# Autodesk Inventor assembly: 15102898-16-A-0300
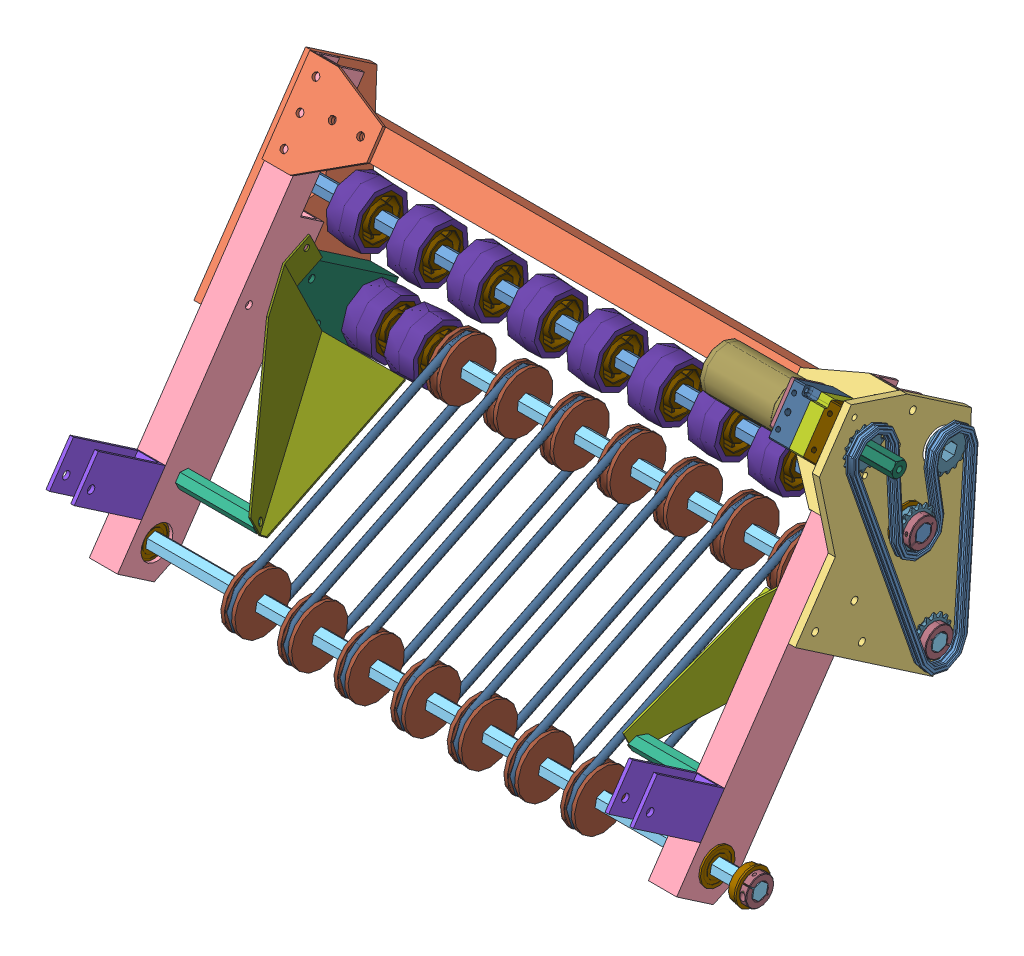
[picture p0: shaded view drawn from the shape stored in the file]
Saved by Autodesk Inventor 2017 (Build 210142000, 142)
## iProperties
Created: 2016-10-02
Part Number: 15102898-16-A-0300
Document SubType Name: Assembly
Designer: gus
Mass: 5609.92 g
Surface Area: 11678.6 cm^2
Volume: 2397.48 cm^3
Density: 2.33992 g/cm^3
Author: gus
## Documents named in this file (23)
- \\Mac\Home\Desktop\bunnybots 2016\15102898-16-Bunnybot-CAD\Bunnybot-To_be_renamed\15102898-16-A-0000\15102898-16-A-0300\15102898-16-A-0300.iam
- \\Mac\Home\Desktop\bunnybots 2016\15102898-16-Bunnybot-CAD\Bunnybot-To_be_renamed\15102898-16-A-0000\15102898-16-A-0300\15102898-16-P-0301.ipt
- \\Mac\Home\Desktop\bunnybots 2016\15102898-16-Bunnybot-CAD\Bunnybot-To_be_renamed\15102898-16-A-0000\15102898-16-A-0300\15102898-16-P-0302.ipt
- \\Mac\Home\Desktop\bunnybots 2016\15102898-16-Bunnybot-CAD\Bunnybot-To_be_renamed\15102898-16-A-0000\15102898-16-A-0300\Imported Components\217-3875-STEP-20140818.ipt
- \\Mac\Home\Desktop\bunnybots 2016\15102898-16-Bunnybot-CAD\Bunnybot-To_be_renamed\15102898-16-A-0000\15102898-16-A-0300\15102898-16-P-0303.ipt
- \\Mac\Home\Desktop\bunnybots 2016\15102898-16-Bunnybot-CAD\Bunnybot-To_be_renamed\15102898-16-A-0000\15102898-16-A-0300\Imported Components\217-2737.20121205.ipt
- \\Mac\Home\Desktop\bunnybots 2016\15102898-16-Bunnybot-CAD\Bunnybot-To_be_renamed\15102898-16-A-0000\15102898-16-A-0300\15102898-16-P-0304.ipt
- \\Mac\Home\Desktop\bunnybots 2016\15102898-16-Bunnybot-CAD\Bunnybot-To_be_renamed\15102898-16-A-0000\15102898-16-A-0300\15102898-16-P-0305.ipt
- \\Mac\Home\Desktop\bunnybots 2016\15102898-16-Bunnybot-CAD\Bunnybot-To_be_renamed\15102898-16-A-0000\15102898-16-A-0300\Imported Components\217-2642-STEP-20140807.ipt
- \\Mac\Home\Desktop\bunnybots 2016\15102898-16-Bunnybot-CAD\Bunnybot-To_be_renamed\15102898-16-A-0000\15102898-16-A-0300\Imported Components\BAG motor\VersaPlanetary-1-Stage-with-BAG-Motor.iam
- \\Mac\Home\Desktop\bunnybots 2016\15102898-16-Bunnybot-CAD\Bunnybot-To_be_renamed\15102898-16-A-0000\15102898-16-A-0300\Imported Components\6284K520_ROUND-BELT PULLEY.ipt
- \\Mac\Home\Desktop\bunnybots 2016\15102898-16-Bunnybot-CAD\Bunnybot-To_be_renamed\15102898-16-A-0000\15102898-16-A-0300\15102898-16-P-0308.ipt
- \\Mac\Home\Desktop\bunnybots 2016\15102898-16-Bunnybot-CAD\Bunnybot-To_be_renamed\15102898-16-A-0000\15102898-16-A-0300\Imported Components\am-3155+2in+Wheel+Intergrated+500+HEX.ipt
- \\Mac\Home\Desktop\bunnybots 2016\15102898-16-Bunnybot-CAD\Bunnybot-To_be_renamed\15102898-16-A-0000\15102898-16-A-0300\15102898-16-P-0307.ipt
- \\Mac\Home\Desktop\bunnybots 2016\15102898-16-Bunnybot-CAD\Bunnybot-To_be_renamed\15102898-16-A-0000\15102898-16-A-0300\15102898-16-P-0309.ipt
- \\Mac\Home\Desktop\bunnybots 2016\15102898-16-Bunnybot-CAD\Bunnybot-To_be_renamed\15102898-16-A-0000\15102898-16-A-0300\15102898-16-P-0310.ipt
- \\Mac\Home\Desktop\bunnybots 2016\15102898-16-Bunnybot-CAD\Bunnybot-To_be_renamed\15102898-16-A-0000\15102898-16-A-0300\15102898-16-A-0311.iam
- \\Mac\Home\Desktop\bunnybots 2016\15102898-16-Bunnybot-CAD\Bunnybot-To_be_renamed\15102898-16-A-0000\15102898-16-A-0300\15102898-16-A-0300\Design Accelerator\Chain Drive2.iam
- \\Mac\Home\Desktop\bunnybots 2016\15102898-16-Bunnybot-CAD\Bunnybot-To_be_renamed\15102898-16-A-0000\15102898-16-A-0300\15102898-16-P-0309_CPY.ipt
- \\Mac\Home\Desktop\bunnybots 2016\15102898-16-Bunnybot-CAD\Bunnybot-To_be_renamed\15102898-16-A-0000\15102898-16-A-0300\15102898-16-P-0311.ipt
- \\Mac\Home\Desktop\bunnybots 2016\15102898-16-Bunnybot-CAD\Bunnybot-To_be_renamed\15102898-16-A-0000\15102898-16-A-0300\15102898-16-P-0312.ipt
- \\Mac\Home\Desktop\bunnybots 2016\15102898-16-Bunnybot-CAD\Bunnybot-To_be_renamed\15102898-16-A-0000\15102898-16-A-0300\15102898-16-P-03121.ipt
- \\Mac\Home\Desktop\bunnybots 2016\15102898-16-Bunnybot-CAD\Bunnybot-To_be_renamed\15102898-16-A-0000\15102898-16-A-0300\15102898-16-P-0314.ipt
## Components (78 placed, 22 different names)
1. 15102898-16-P-0301:1 — Flush:1, Flush:2, Mate:1, Flush:3, Mate:3, Mate:14, Flush:8, Flush:11, Flush:18, Flush:19, Flush:33, Mate:97, Flush:36, Flush:37, Mate:98, Mate:105, Mate:109, Mate:110, Mate:111, Flush:46, Mate:116, Mate:128, Mate:131, Mate:133
2. 15102898-16-P-0301:2 — Flush:1, Flush:2, Mate:3, Mate:15, Flush:14, Mate:96, Flush:34, Mate:100, Flush:38, Mate:101, Flush:40, Flush:41, Mate:112, Mate:113, Flush:48, Mate:117, Angle:1, Mate:121, Symmetry:1, Mate:130
3. 15102898-16-P-0302:1 — Mate:1, Flush:3, Cylindrical:1, Mate:5, Flush:19, Mate:52, Mate:54, Flush:39
4. 217-3875-STEP-20140818:1 — Mate:13
5. 217-3875-STEP-20140818:2 — Cylindrical:1, Mate:5, Mate:6, Mate:7, Mate:49, Mate:50
6. 15102898-16-P-0303:1 — Mate:6, Mate:7, Mate:8, Mate:9, Mate:11, Mate:12, Flush:7, Mate:94, Mate:95
7. 217-2737.20121205:1 — Mate:11, Mate:12, Mate:13
8. 217-2737.20121205:2 — Mate:8, Mate:9, Flush:7, Mate:55
9. 15102898-16-P-0304:1 — Mate:14, Flush:8, Mate:16, Flush:11, Flush:13
10. 15102898-16-P-0304:2 — Mate:15, Flush:13, Flush:14, Cylindrical:8, Mate:29, Mate:74, Mate:83
11. 217-3875-STEP-20140818:3 — Mate:16, Mate:19, Mate:20, Mate:47, Mate:48
12. 15102898-16-P-0305:1 — Mate:19, Mate:20, Flush:12, Mate:23, Mate:24, Mate:57, Mate:58, Mate:70, Mate:71, Mate:81, Mate:82, Mate:84, Mate:85, Mate:91, Mate:92, Mate:119, Mate:136
13. 217-2737.20121205:3 — Flush:12, Mate:23, Mate:24, Mate:53
14. 217-3875-STEP-20140818:6 — Cylindrical:8, Mate:29, Mate:56
15. 217-2737.20121205:4 — Mate:56, Mate:57, Mate:58, Mate:115
16. VersaPlanetary-1-Stage-with-BAG-Motor:1 [sub-assembly] — Flush:18, Mate:45, Mate:46, Flush:33, Flush:35, Mate:99
17. 217-2642-STEP-20140807:4 — Mate:45, Mate:46
18. 217-2642-STEP-20140807:5 — Mate:47, Mate:48, Mate:53
19. 217-2642-STEP-20140807:6 — Mate:49, Mate:50, Mate:55
20. 217-2642-STEP-20140807:7 — Mate:52, Mate:54
21. 217-3875-STEP-20140818:7 — Mate:64, Mate:65, Mate:69, Mate:105, Mate:109
22. 217-3875-STEP-20140818:8 — Mate:66, Flush:45, Mate:106
23. 15102898-16-P-0305:2 — Mate:64, Mate:65, Mate:66, Flush:26, Mate:67, Mate:68, Mate:72, Mate:73, Flush:45, Mate:106, Mate:114
24. 217-2737.20121205:5 — Flush:26, Mate:67, Mate:68, Mate:69
25. am-3155+2in+Wheel+Intergrated+500+HEX:1 — Mate:81, Mate:82, Mate:83, Mate:86
26. am-3155+2in+Wheel+Intergrated+500+HEX:2 — Mate:84, Mate:85, Mate:86
27. 15102898-16-P-0307:1 — Flush:34, Mate:97, Flush:35
28. 15102898-16-P-0309:1 — Flush:36, Flush:37, Mate:98, Mate:99
29. 15102898-16-P-0310:1 — Mate:100, Flush:38, Flush:39, Mate:115
30. 15102898-16-A-0311:1 [sub-assembly]
31. Chain Drive:1 [sub-assembly]
32. 15102898-16-P-0309_CPY:1 — Mate:101, Flush:40, Flush:41
33. 217-3875-STEP-20140818:9 — Mate:110, Mate:111, Mate:114
34. 217-3875-STEP-20140818:10 — Mate:112, Mate:113
35. 15102898-16-P-0311:1 — Flush:46, Mate:116, Flush:49, Symmetry:1, Mate:133
36. 15102898-16-P-0311:2 — Flush:48, Mate:117, Flush:49
37. 15102898-16-P-0312:1 — Angle:1, Tangent:2, Angle:2, Mate:120, Mate:121, Flush:54, Flush:55
38. 15102898-16-P-03121:1 — Mate:124, Flush:54, Flush:55, Mate:128, Mate:132
39. 15102898-16-P-0314:1 — Mate:129, Flush:56, Mate:131, Mate:132
40. 15102898-16-P-0314:2 — Mate:129, Flush:56, Mate:130
41. am-3155+2in+Wheel+Intergrated+500+HEX:26 — Mate:135, Mate:136, Mate:137, Mate:138, Mate:139
42. am-3155+2in+Wheel+Intergrated+500+HEX:27 — Mate:138, Mate:139
43. 6284K520_ROUND-BELT PULLEY:1 — Mate:70, Mate:71, Flush:28, Mate:74, Mate:107, Tangent:1
44. 6284K520_ROUND-BELT PULLEY:2 — Mate:93
45. 6284K520_ROUND-BELT PULLEY:3
46. 6284K520_ROUND-BELT PULLEY:4
47. 6284K520_ROUND-BELT PULLEY:5
48. 6284K520_ROUND-BELT PULLEY:6
49. 6284K520_ROUND-BELT PULLEY:7
50. 6284K520_ROUND-BELT PULLEY:10 — Mate:72, Mate:73, Flush:28, Mate:108
51. 6284K520_ROUND-BELT PULLEY:11
52. 6284K520_ROUND-BELT PULLEY:12
53. 6284K520_ROUND-BELT PULLEY:13
54. 6284K520_ROUND-BELT PULLEY:14
55. 6284K520_ROUND-BELT PULLEY:15
56. 6284K520_ROUND-BELT PULLEY:16
57. 15102898-16-P-0308:1 — Mate:107, Mate:108, Tangent:1, Tangent:2
58. 15102898-16-P-0308:2
59. 15102898-16-P-0308:3
60. 15102898-16-P-0308:4
61. 15102898-16-P-0308:5
62. 15102898-16-P-0308:6
63. 15102898-16-P-0308:7
64. am-3155+2in+Wheel+Intergrated+500+HEX:11 — Mate:94, Mate:95, Mate:96
65. am-3155+2in+Wheel+Intergrated+500+HEX:12
66. am-3155+2in+Wheel+Intergrated+500+HEX:13
67. am-3155+2in+Wheel+Intergrated+500+HEX:14
68. am-3155+2in+Wheel+Intergrated+500+HEX:15
69. am-3155+2in+Wheel+Intergrated+500+HEX:16
70. am-3155+2in+Wheel+Intergrated+500+HEX:17
71. am-3155+2in+Wheel+Intergrated+500+HEX:18
72. am-3155+2in+Wheel+Intergrated+500+HEX:19
73. am-3155+2in+Wheel+Intergrated+500+HEX:5 — Mate:91, Mate:92, Mate:93
74. am-3155+2in+Wheel+Intergrated+500+HEX:20
75. am-3155+2in+Wheel+Intergrated+500+HEX:21
76. am-3155+2in+Wheel+Intergrated+500+HEX:22
77. am-3155+2in+Wheel+Intergrated+500+HEX:23
78. am-3155+2in+Wheel+Intergrated+500+HEX:24 — Mate:135, Mate:137
## Component patterns: (7 elements, first: 6284K520_ROUND-BELT PULLEY:1), (7 elements, first: 6284K520_ROUND-BELT PULLEY:10), (7 elements, first: 15102898-16-P-0308:1), (9 elements, first: am-3155+2in+Wheel+Intergrated+500+HEX:11), (6 elements, first: am-3155+2in+Wheel+Intergrated+500+HEX:5)
## Relationships (125: Mate 87, Flush 31, CylindricalJoint 2, Tangent 2, Angle 2, Symmetry 1)
- Flush:1: 15102898-16-P-0301:1 ↔ 15102898-16-P-0301:2
- Flush:2: 15102898-16-P-0301:1 ↔ 15102898-16-P-0301:2
- Mate:1: 15102898-16-P-0301:1 ↔ 15102898-16-P-0302:1
- Flush:3: 15102898-16-P-0301:1 ↔ 15102898-16-P-0302:1
- Mate:3 (476.25 mm): 15102898-16-P-0301:1 ↔ 15102898-16-P-0301:2
- Cylindrical:1: 15102898-16-P-0302:1 ↔ 217-3875-STEP-20140818:2
- Mate:5: 15102898-16-P-0302:1 ↔ 217-3875-STEP-20140818:2
- Mate:6: 217-3875-STEP-20140818:2 ↔ 15102898-16-P-0303:1
- Mate:7: 217-3875-STEP-20140818:2 ↔ 15102898-16-P-0303:1
- Mate:8: 15102898-16-P-0303:1 ↔ 217-2737.20121205:2
- Mate:9: 15102898-16-P-0303:1 ↔ 217-2737.20121205:2
- Mate:11: 15102898-16-P-0303:1 ↔ 217-2737.20121205:1
- Mate:12: 15102898-16-P-0303:1 ↔ 217-2737.20121205:1
- Mate:13: 217-3875-STEP-20140818:1 ↔ 217-2737.20121205:1
- Flush:7: 15102898-16-P-0303:1 ↔ 217-2737.20121205:2
- Mate:14: 15102898-16-P-0301:1 ↔ 15102898-16-P-0304:1
- Flush:8: 15102898-16-P-0301:1 ↔ 15102898-16-P-0304:1
- Mate:15: 15102898-16-P-0301:2 ↔ 15102898-16-P-0304:2
- Mate:16: 15102898-16-P-0304:1 ↔ 217-3875-STEP-20140818:3
- Mate:19: 217-3875-STEP-20140818:3 ↔ 15102898-16-P-0305:1
- Mate:20: 217-3875-STEP-20140818:3 ↔ 15102898-16-P-0305:1
- Flush:11 (127 mm): 15102898-16-P-0301:1 ↔ 15102898-16-P-0304:1
- Flush:12: 15102898-16-P-0305:1 ↔ 217-2737.20121205:3
- Mate:23: 15102898-16-P-0305:1 ↔ 217-2737.20121205:3
- Mate:24: 15102898-16-P-0305:1 ↔ 217-2737.20121205:3
- Flush:13: 15102898-16-P-0304:1 ↔ 15102898-16-P-0304:2
- Flush:14: 15102898-16-P-0301:2 ↔ 15102898-16-P-0304:2
- Cylindrical:8: 15102898-16-P-0304:2 ↔ 217-3875-STEP-20140818:6
- Mate:29: 15102898-16-P-0304:2 ↔ 217-3875-STEP-20140818:6
- Flush:18: 15102898-16-P-0301:1 ↔ VersaPlanetary-1-Stage-with-BAG-Motor:1
- Mate:45: VersaPlanetary-1-Stage-with-BAG-Motor:1 ↔ 217-2642-STEP-20140807:4
- Mate:46: VersaPlanetary-1-Stage-with-BAG-Motor:1 ↔ 217-2642-STEP-20140807:4
- Mate:47: 217-3875-STEP-20140818:3 ↔ 217-2642-STEP-20140807:5
- Mate:48: 217-3875-STEP-20140818:3 ↔ 217-2642-STEP-20140807:5
- Mate:49: 217-3875-STEP-20140818:2 ↔ 217-2642-STEP-20140807:6
- Mate:50: 217-3875-STEP-20140818:2 ↔ 217-2642-STEP-20140807:6
- Mate:52: 15102898-16-P-0302:1 ↔ 217-2642-STEP-20140807:7
- Flush:19: 15102898-16-P-0301:1 ↔ 15102898-16-P-0302:1
- Mate:53: 217-2737.20121205:3 ↔ 217-2642-STEP-20140807:5
- Mate:54: 15102898-16-P-0302:1 ↔ 217-2642-STEP-20140807:7
- Mate:55: 217-2737.20121205:2 ↔ 217-2642-STEP-20140807:6
- Mate:56: 217-3875-STEP-20140818:6 ↔ 217-2737.20121205:4
- Mate:57: 15102898-16-P-0305:1 ↔ 217-2737.20121205:4
- Mate:58: 15102898-16-P-0305:1 ↔ 217-2737.20121205:4
- Mate:64: 217-3875-STEP-20140818:7 ↔ 15102898-16-P-0305:2
- Mate:65: 217-3875-STEP-20140818:7 ↔ 15102898-16-P-0305:2
- Mate:66: 217-3875-STEP-20140818:8 ↔ 15102898-16-P-0305:2
- Flush:26: 15102898-16-P-0305:2 ↔ 217-2737.20121205:5
- Mate:67: 15102898-16-P-0305:2 ↔ 217-2737.20121205:5
- Mate:68: 15102898-16-P-0305:2 ↔ 217-2737.20121205:5
- Mate:69: 217-3875-STEP-20140818:7 ↔ 217-2737.20121205:5
- Mate:70: 15102898-16-P-0305:1 ↔ 6284K520_ROUND-BELT PULLEY:1
- Mate:71: 15102898-16-P-0305:1 ↔ 6284K520_ROUND-BELT PULLEY:1
- Mate:72: 15102898-16-P-0305:2 ↔ 6284K520_ROUND-BELT PULLEY:10
- Mate:73: 15102898-16-P-0305:2 ↔ 6284K520_ROUND-BELT PULLEY:10
- Flush:28: 6284K520_ROUND-BELT PULLEY:1 ↔ 6284K520_ROUND-BELT PULLEY:10
- Mate:74 (82.55 mm): 15102898-16-P-0304:2 ↔ 6284K520_ROUND-BELT PULLEY:1
- Mate:81: 15102898-16-P-0305:1 ↔ am-3155+2in+Wheel+Intergrated+500+HEX:1
- Mate:82: 15102898-16-P-0305:1 ↔ am-3155+2in+Wheel+Intergrated+500+HEX:1
- Mate:83 (6.35 mm): 15102898-16-P-0304:2 ↔ am-3155+2in+Wheel+Intergrated+500+HEX:1
- Mate:84: 15102898-16-P-0305:1 ↔ am-3155+2in+Wheel+Intergrated+500+HEX:2
- Mate:85: 15102898-16-P-0305:1 ↔ am-3155+2in+Wheel+Intergrated+500+HEX:2
- Mate:86 (12.7 mm): am-3155+2in+Wheel+Intergrated+500+HEX:1 ↔ am-3155+2in+Wheel+Intergrated+500+HEX:2
- Mate:91: 15102898-16-P-0305:1 ↔ am-3155+2in+Wheel+Intergrated+500+HEX:5
- Mate:92: 15102898-16-P-0305:1 ↔ am-3155+2in+Wheel+Intergrated+500+HEX:5
- Mate:93 (6.35 mm): 6284K520_ROUND-BELT PULLEY:2 ↔ am-3155+2in+Wheel+Intergrated+500+HEX:5
- Mate:94: 15102898-16-P-0303:1 ↔ am-3155+2in+Wheel+Intergrated+500+HEX:11
- Mate:95: 15102898-16-P-0303:1 ↔ am-3155+2in+Wheel+Intergrated+500+HEX:11
- Mate:96 (12.7 mm): 15102898-16-P-0301:2 ↔ am-3155+2in+Wheel+Intergrated+500+HEX:11
- Flush:33 (19.05 mm): 15102898-16-P-0301:1 ↔ VersaPlanetary-1-Stage-with-BAG-Motor:1
- Flush:34: 15102898-16-P-0301:2 ↔ 15102898-16-P-0307:1
- Mate:97: 15102898-16-P-0301:1 ↔ 15102898-16-P-0307:1
- Flush:35: VersaPlanetary-1-Stage-with-BAG-Motor:1 ↔ 15102898-16-P-0307:1
- Flush:36: 15102898-16-P-0301:1 ↔ 15102898-16-P-0309:1
- Flush:37: 15102898-16-P-0301:1 ↔ 15102898-16-P-0309:1
- Mate:98: 15102898-16-P-0301:1 ↔ 15102898-16-P-0309:1
- Mate:99: VersaPlanetary-1-Stage-with-BAG-Motor:1 ↔ 15102898-16-P-0309:1
- Mate:100: 15102898-16-P-0301:2 ↔ 15102898-16-P-0310:1
- Flush:38: 15102898-16-P-0301:2 ↔ 15102898-16-P-0310:1
- Flush:39: 15102898-16-P-0302:1 ↔ 15102898-16-P-0310:1
- Mate:101: 15102898-16-P-0301:2 ↔ 15102898-16-P-0309_CPY:1
- Flush:40: 15102898-16-P-0301:2 ↔ 15102898-16-P-0309_CPY:1
- Flush:41: 15102898-16-P-0301:2 ↔ 15102898-16-P-0309_CPY:1
- Mate:105: 15102898-16-P-0301:1 ↔ 217-3875-STEP-20140818:7
- Flush:45 (6.35 mm): 217-3875-STEP-20140818:8 ↔ 15102898-16-P-0305:2
- Mate:106: 217-3875-STEP-20140818:8 ↔ 15102898-16-P-0305:2
- Mate:107: 6284K520_ROUND-BELT PULLEY:1 ↔ 15102898-16-P-0308:1
- Mate:108: 6284K520_ROUND-BELT PULLEY:10 ↔ 15102898-16-P-0308:1
- Tangent:1: 6284K520_ROUND-BELT PULLEY:1 ↔ 15102898-16-P-0308:1
- Mate:109 (25.4 mm): 15102898-16-P-0301:1 ↔ 217-3875-STEP-20140818:7
- Mate:110: 15102898-16-P-0301:1 ↔ 217-3875-STEP-20140818:9
- Mate:111: 15102898-16-P-0301:1 ↔ 217-3875-STEP-20140818:9
- Mate:112: 15102898-16-P-0301:2 ↔ 217-3875-STEP-20140818:10
- Mate:113: 15102898-16-P-0301:2 ↔ 217-3875-STEP-20140818:10
- Mate:114: 15102898-16-P-0305:2 ↔ 217-3875-STEP-20140818:9
- Mate:115: 217-2737.20121205:4 ↔ 15102898-16-P-0310:1
- Flush:46: 15102898-16-P-0301:1 ↔ 15102898-16-P-0311:1
- Mate:116: 15102898-16-P-0301:1 ↔ 15102898-16-P-0311:1
- Flush:48: 15102898-16-P-0301:2 ↔ 15102898-16-P-0311:2
- Mate:117: 15102898-16-P-0301:2 ↔ 15102898-16-P-0311:2
- Flush:49: 15102898-16-P-0311:1 ↔ 15102898-16-P-0311:2
- Angle:1 (0 deg): 15102898-16-P-0301:2 ↔ 15102898-16-P-0312:1
- Tangent:2: 15102898-16-P-0312:1 ↔ 15102898-16-P-0308:1
- Mate:119: 15102898-16-P-0305:1
- Angle:2 (0 deg): 15102898-16-P-0312:1
- Flush:50 (-25.4 mm)
- Mate:120: 15102898-16-P-0312:1
- Mate:121: 15102898-16-P-0301:2 ↔ 15102898-16-P-0312:1
- Symmetry:1: 15102898-16-P-0301:2 ↔ 15102898-16-P-0311:1
- Mate:124: 15102898-16-P-03121:1
- Flush:51 (-25.4 mm)
- Flush:54: 15102898-16-P-0312:1 ↔ 15102898-16-P-03121:1
- Flush:55: 15102898-16-P-0312:1 ↔ 15102898-16-P-03121:1
- Mate:128: 15102898-16-P-0301:1 ↔ 15102898-16-P-03121:1
- Mate:129: 15102898-16-P-0314:1 ↔ 15102898-16-P-0314:2
- Flush:56: 15102898-16-P-0314:1 ↔ 15102898-16-P-0314:2
- Mate:130: 15102898-16-P-0301:2 ↔ 15102898-16-P-0314:2
- Mate:131: 15102898-16-P-0301:1 ↔ 15102898-16-P-0314:1
- Mate:132: 15102898-16-P-03121:1 ↔ 15102898-16-P-0314:1
- Mate:133 (-76.2 mm): 15102898-16-P-0301:1 ↔ 15102898-16-P-0311:1
- Mate:135 (25.4 mm): am-3155+2in+Wheel+Intergrated+500+HEX:26 ↔ am-3155+2in+Wheel+Intergrated+500+HEX:24
- Mate:136: 15102898-16-P-0305:1 ↔ am-3155+2in+Wheel+Intergrated+500+HEX:26
- Mate:137: am-3155+2in+Wheel+Intergrated+500+HEX:26 ↔ am-3155+2in+Wheel+Intergrated+500+HEX:24
- Mate:138 (25.4 mm): am-3155+2in+Wheel+Intergrated+500+HEX:26 ↔ am-3155+2in+Wheel+Intergrated+500+HEX:27
- Mate:139: am-3155+2in+Wheel+Intergrated+500+HEX:26 ↔ am-3155+2in+Wheel+Intergrated+500+HEX:27
